# Autodesk Inventor assembly: TAD
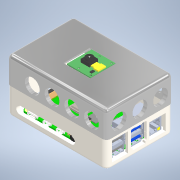
[picture p0: Inventor's stored thumbnail of the model, 180x180]
Saved by Autodesk Inventor 2021 (Build 250183000, 183)
## iProperties
Created: 2022-12-30
Part Number: TAD
Document SubType Name: Assembly
Designer: Nihal
Author: Nihal
## Documents named in this file (5)
- C:\Users\Nihal\Desktop\thermal-anomaly-detection\cad\TAD.iam
- C:\Users\Nihal\Desktop\thermal-anomaly-detection\cad\Plastic Case.ipt
- C:\Users\Nihal\Desktop\thermal-anomaly-detection\cad\Raspberry Pi 4 Model B.iam
- C:\Users\Nihal\Desktop\thermal-anomaly-detection\cad\RPi cam Rev 1.3.ipt
- C:\Users\Nihal\Desktop\thermal-anomaly-detection\cad\TopCover.ipt
## Components (4 placed, 4 different names)
1. Plastic Case:1 — Mate:1, Mate:2, Mate:3, Mate:5, Flush:1, Flush:2
2. Raspberry Pi 4 Model B:1 [sub-assembly] — Mate:1, Mate:2, Mate:3
3. RPi cam Rev 1.3:1 — Mate:6
4. TopCover:1 — Mate:5, Flush:1, Flush:2, Mate:6
## Relationships (7: Mate 5, Flush 2)
- Mate:1: Plastic Case:1 ↔ Raspberry Pi 4 Model B:1
- Mate:2: Plastic Case:1 ↔ Raspberry Pi 4 Model B:1
- Mate:3: Plastic Case:1 ↔ Raspberry Pi 4 Model B:1
- Mate:5: Plastic Case:1 ↔ TopCover:1
- Flush:1: Plastic Case:1 ↔ TopCover:1
- Flush:2: Plastic Case:1 ↔ TopCover:1
- Mate:6: RPi cam Rev 1.3:1 ↔ TopCover:1
